# Autodesk Inventor assembly: 付け根_1
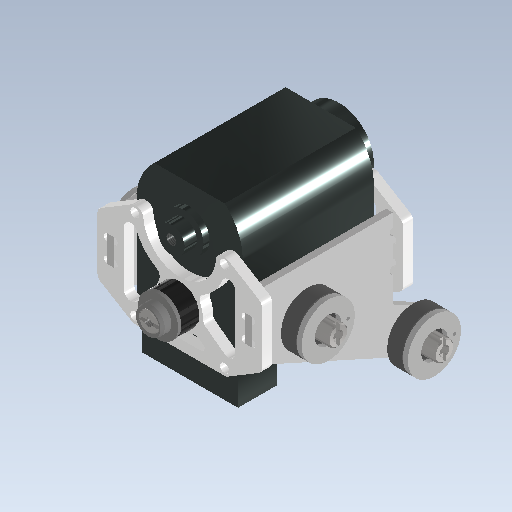
[picture p0: Inventor's stored thumbnail of the model, 512x512]
Saved by Autodesk Inventor 2020 (Build 240168000, 168)
## iProperties
Created: 2021-09-06
Part Number: 付け根_1
Document SubType Name: Assembly
Designer: Masato
Mass: 128.277 g
Surface Area: 254.219 cm^2
Volume: 69.2239 cm^3
Density: 1.85308 g/cm^3
Author: Masato
## Documents named in this file (13)
- C:\Users\Masato\Desktop\最新版\OpenPlatform_ver3_0\下半身\付け根\付け根_1.iam
- C:\Users\Masato\Desktop\最新版\OpenPlatform_ver3_0\下半身\付け根\付け根_メインフレーム_1.ipt
- C:\Users\Masato\Desktop\最新版\OpenPlatform_ver3_0\下半身\付け根\付け根_メインフレーム_6_1.ipt
- C:\Users\Masato\Desktop\最新版\OpenPlatform_ver3_0\Ready_Made\B3M11xx.ipt
- C:\Users\Masato\Desktop\最新版\OpenPlatform_ver3_0\Ready_Made\SLSBF6-39_5-M3-N3.ipt
- C:\Users\Masato\Desktop\最新版\OpenPlatform_ver3_0\Ready_Made\ARU-3010S.ipt
- C:\Users\Masato\Desktop\最新版\OpenPlatform_ver3_0\Ready_Made\CC-0612-25B.ipt
- C:\Users\Masato\Desktop\最新版\OpenPlatform_ver3_0\Ready_Made\CC-0612-30B.ipt
- C:\Users\Masato\Desktop\最新版\OpenPlatform_ver3_0\Ready_Made\80F-0603.ipt
- C:\Users\Masato\Desktop\最新版\OpenPlatform_ver3_0\Ready_Made\UUW-0312-10BH.ipt
- C:\Users\Masato\Desktop\最新版\OpenPlatform_ver3_0\Ready_Made\BRU-309_5S.ipt
- C:\Users\Masato\Desktop\最新版\OpenPlatform_ver3_0\Ready_Made\GSB-081605.ipt
- C:\Users\Masato\Desktop\最新版\OpenPlatform_ver3_0\Ready_Made\LFW-0815.ipt
## Components (30 placed, 12 different names)
1. 付け根_メインフレーム_1:1 — メイト:1, メイト:2, フラッシュ:1, 挿入:11, 挿入:27, 挿入:28
2. 付け根_メインフレーム_1:2 — メイト:3, メイト:4, フラッシュ:2, 挿入:12, 挿入:25, 挿入:26
3. 付け根_メインフレーム_6_1:1 — 挿入:3, 挿入:4, 挿入:5, 挿入:6, メイト:1, メイト:2, フラッシュ:1, メイト:3, メイト:4, フラッシュ:2, 挿入:13
4. 付け根_メインフレーム_6_1:2 — 挿入:7, 挿入:8, 挿入:9, 挿入:10, 挿入:14
5. B3M11xx:1 — 挿入:3, 挿入:4, 挿入:5, 挿入:6, 挿入:7, 挿入:8, 挿入:9, 挿入:10, フラッシュ:6, メイト:8
6. SLSBF6-39_5-M3-N3:1 — 挿入:11, 挿入:12
7. ARU-3010:1 — 挿入:14, 挿入:23
8. ARU-3010:2 — 挿入:13, 挿入:21
9. CC-0612-25B:1 — 挿入:21, 挿入:22
10. CC-0612-30B:1 — 挿入:19, 挿入:22
11. CC-0612-25B:2 — 挿入:23, 挿入:24
12. CC-0612-30B:2 — 挿入:20, 挿入:24
13. 80F-0603:1 — 挿入:19
14. 80F-0603:2 — 挿入:20
15. UUW-0312-10BH:1 — 挿入:27, 挿入:35, 挿入:37
16. UUW-0312-10BH:2 — 挿入:28, 挿入:33, 挿入:38
17. UUW-0312-10BH:3 — 挿入:25, 挿入:36, 挿入:39
18. UUW-0312-10BH:4 — 挿入:26, 挿入:34, 挿入:40
19. BRU-309_5S:1 — 挿入:33
20. BRU-309_5S:2 — 挿入:34
21. BRU-309_5S:3 — 挿入:35
22. BRU-309_5S:4 — 挿入:36
23. GSB-081605:1 — 挿入:37, 挿入:41
24. GSB-081605:2 — 挿入:39, 挿入:44
25. GSB-081605:3 — 挿入:40, 挿入:43
26. GSB-081605:4 — 挿入:38, 挿入:42
27. LFW-0815:1 — 挿入:43
28. LFW-0815:2 — 挿入:44
29. LFW-0815:3 — 挿入:42
30. LFW-0815:4 — 挿入:41
## Relationships (42: Insert 34, Mate 5, Flush 3)
- 挿入:3 [Insert]: 付け根_メインフレーム_6_1:1 ↔ B3M11xx:1
- 挿入:4 [Insert]: 付け根_メインフレーム_6_1:1 ↔ B3M11xx:1
- 挿入:5 [Insert]: 付け根_メインフレーム_6_1:1 ↔ B3M11xx:1
- 挿入:6 [Insert]: 付け根_メインフレーム_6_1:1 ↔ B3M11xx:1
- 挿入:7 [Insert]: 付け根_メインフレーム_6_1:2 ↔ B3M11xx:1
- 挿入:8 [Insert]: 付け根_メインフレーム_6_1:2 ↔ B3M11xx:1
- 挿入:9 [Insert]: 付け根_メインフレーム_6_1:2 ↔ B3M11xx:1
- 挿入:10 [Insert]: 付け根_メインフレーム_6_1:2 ↔ B3M11xx:1
- メイト:1 [Mate] (0.01 mm): 付け根_メインフレーム_1:1 ↔ 付け根_メインフレーム_6_1:1
- メイト:2 [Mate] (0.01 mm): 付け根_メインフレーム_1:1 ↔ 付け根_メインフレーム_6_1:1
- フラッシュ:1 [Flush]: 付け根_メインフレーム_1:1 ↔ 付け根_メインフレーム_6_1:1
- メイト:3 [Mate] (0.01 mm): 付け根_メインフレーム_1:2 ↔ 付け根_メインフレーム_6_1:1
- メイト:4 [Mate] (0.01 mm): 付け根_メインフレーム_1:2 ↔ 付け根_メインフレーム_6_1:1
- フラッシュ:2 [Flush]: 付け根_メインフレーム_1:2 ↔ 付け根_メインフレーム_6_1:1
- 挿入:11 [Insert]: 付け根_メインフレーム_1:1 ↔ SLSBF6-39_5-M3-N3:1
- 挿入:12 [Insert]: 付け根_メインフレーム_1:2 ↔ SLSBF6-39_5-M3-N3:1
- 挿入:13 [Insert]: 付け根_メインフレーム_6_1:1 ↔ ARU-3010:2
- 挿入:14 [Insert]: 付け根_メインフレーム_6_1:2 ↔ ARU-3010:1
- 挿入:19 [Insert]: CC-0612-30B:1 ↔ 80F-0603:1
- 挿入:20 [Insert]: CC-0612-30B:2 ↔ 80F-0603:2
- 挿入:21 [Insert]: ARU-3010:2 ↔ CC-0612-25B:1
- 挿入:22 [Insert]: CC-0612-25B:1 ↔ CC-0612-30B:1
- 挿入:23 [Insert]: ARU-3010:1 ↔ CC-0612-25B:2
- 挿入:24 [Insert]: CC-0612-25B:2 ↔ CC-0612-30B:2
- 挿入:25 [Insert]: 付け根_メインフレーム_1:2 ↔ UUW-0312-10BH:3
- 挿入:26 [Insert]: 付け根_メインフレーム_1:2 ↔ UUW-0312-10BH:4
- 挿入:27 [Insert]: 付け根_メインフレーム_1:1 ↔ UUW-0312-10BH:1
- 挿入:28 [Insert]: 付け根_メインフレーム_1:1 ↔ UUW-0312-10BH:2
- 挿入:33 [Insert]: UUW-0312-10BH:2 ↔ BRU-309_5S:1
- 挿入:34 [Insert]: UUW-0312-10BH:4 ↔ BRU-309_5S:2
- フラッシュ:6 [Flush]: B3M11xx:1
- メイト:8 [Mate]: B3M11xx:1
- 挿入:35 [Insert]: UUW-0312-10BH:1 ↔ BRU-309_5S:3
- 挿入:36 [Insert]: UUW-0312-10BH:3 ↔ BRU-309_5S:4
- 挿入:37 [Insert]: UUW-0312-10BH:1 ↔ GSB-081605:1
- 挿入:38 [Insert]: UUW-0312-10BH:2 ↔ GSB-081605:4
- 挿入:39 [Insert]: UUW-0312-10BH:3 ↔ GSB-081605:2
- 挿入:40 [Insert]: UUW-0312-10BH:4 ↔ GSB-081605:3
- 挿入:41 [Insert]: GSB-081605:1 ↔ LFW-0815:4
- 挿入:42 [Insert]: GSB-081605:4 ↔ LFW-0815:3
- 挿入:43 [Insert]: GSB-081605:3 ↔ LFW-0815:1
- 挿入:44 [Insert]: GSB-081605:2 ↔ LFW-0815:2
